# Autodesk Inventor assembly: Table
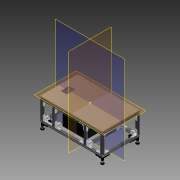
[picture p0: Inventor's stored thumbnail of the model, 180x180]
Saved by Autodesk Inventor 2015 (Build 190159000, 159)
## iProperties
Created: 2015-12-24
Part Number: Table
Document SubType Name: Assembly
Designer: Ryo
Author: Ryo
## Documents named in this file (10)
- D:\Users\Ryo\Documents\Inventor\motoman_cad\SIA5_TABLE\INVENTOR2015\Table_no_bis.iam
- D:\Users\Ryo\Documents\Inventor\motoman_table\EFS8-4040-580.ipt
- D:\Users\Ryo\Documents\Inventor\motoman_table\EFS8-4040-305.ipt
- D:\Users\Ryo\Documents\Inventor\motoman_cad\SIA5_TABLE\parts\EFS8-4040-1100.ipt
- D:\Users\Ryo\Documents\Inventor\motoman_cad\SIA5_TABLE\parts\SFK-N19T.ipt
- D:\Users\Ryo\Documents\Inventor\motoman_cad\SIA5_TABLE\INVENTOR2015\board.ipt
- D:\Users\Ryo\Documents\Inventor\motoman_cad\SIA5_TABLE\INVENTOR2015\controller_table.ipt
- D:\Users\Ryo\Documents\Inventor\motoman_cad\SIA5_TABLE\INVENTOR2015\controller.ipt
- D:\Users\Ryo\Documents\Inventor\Content Center Files\R2015\ja-JP\JIS B 1176\JIS B 1176 - M6 x 10.ipt
- D:\Users\Ryo\Documents\Inventor\motoman_cad\SIA5_TABLE\INVENTOR2015\foot_parts.iam
## Components (101 placed, 9 different names)
1. EFS8-4040-580:1 — フラッシュ:63, フラッシュ:64, メイト:70, フラッシュ:82, メイト:81, メイト:85, メイト:89, フラッシュ:86, メイト:91, フラッシュ:114
2. EFS8-4040-580:2 — フラッシュ:43, フラッシュ:44, メイト:44, フラッシュ:47, メイト:47, フラッシュ:49, メイト:51, フラッシュ:83, メイト:83, フラッシュ:89, メイト:95, フラッシュ:119, フラッシュ:122
3. EFS8-4040-580:4 — フラッシュ:16, メイト:26, フラッシュ:17, フラッシュ:18, フラッシュ:20, フラッシュ:54, メイト:62, フラッシュ:77, フラッシュ:78, フラッシュ:98, メイト:114, メイト:116, メイト:133
4. EFS8-4040-580:5 — フラッシュ:74, フラッシュ:75, メイト:73, フラッシュ:76, フラッシュ:95, メイト:108, フラッシュ:96, メイト:109, フラッシュ:101, メイト:119, フラッシュ:102, メイト:121
5. EFS8-4040-580:6 — フラッシュ:1, メイト:14, フラッシュ:2, フラッシュ:3, メイト:15, フラッシュ:4, フラッシュ:13, メイト:20, フラッシュ:15, メイト:24, フラッシュ:74, メイト:112, フラッシュ:100, メイト:117, フラッシュ:116, メイト:308, フラッシュ:118, メイト:309
6. EFS8-4040-580:7 — フラッシュ:68, メイト:72, フラッシュ:76, メイト:135, メイト:138, フラッシュ:111, メイト:140, フラッシュ:112, メイト:142
7. EFS8-4040-580:8 — フラッシュ:45, フラッシュ:46, メイト:45, フラッシュ:48, メイト:49, メイト:58, フラッシュ:52, メイト:74, フラッシュ:90, メイト:98, フラッシュ:91, メイト:100
8. EFS8-4040-305:1 — フラッシュ:18, フラッシュ:19, メイト:27, メイト:63, メイト:64, メイト:66, メイト:101, メイト:104
9. EFS8-4040-305:2 — フラッシュ:5, フラッシュ:6, メイト:16, メイト:18, フラッシュ:11, メイト:21, メイト:105, メイト:107
10. EFS8-4040-305:3 — フラッシュ:20, フラッシュ:21, メイト:28, メイト:34, メイト:36, フラッシュ:104, メイト:125, フラッシュ:105, メイト:128, メイト:134, フラッシュ:108
11. EFS8-4040-305:4 — フラッシュ:28, フラッシュ:29, メイト:32, メイト:42, メイト:46, フラッシュ:61, メイト:69, フラッシュ:62, メイト:90, メイト:94
12. EFS8-4040-305:5 — フラッシュ:7, フラッシュ:8, フラッシュ:9, メイト:17, メイト:22, メイト:25, メイト:120, フラッシュ:103, メイト:124
13. EFS8-4040-305:6 — フラッシュ:24, フラッシュ:25, メイト:30, フラッシュ:45, メイト:57, メイト:59, メイト:60, メイト:79, メイト:87
14. EFS8-4040-305:7 — フラッシュ:26, フラッシュ:27, メイト:31, メイト:50, メイト:52, メイト:54, フラッシュ:59, フラッシュ:60, メイト:68, メイト:78, メイト:82
15. EFS8-4040-305:8 — フラッシュ:22, フラッシュ:23, メイト:29, メイト:38, メイト:39, メイト:48, メイト:129, メイト:132
16. EFS8-4040-1100:1 — フラッシュ:3, メイト:15, フラッシュ:4, フラッシュ:7, フラッシュ:8, フラッシュ:9, メイト:17, フラッシュ:14, メイト:23, メイト:26, フラッシュ:17, フラッシュ:21, メイト:28, フラッシュ:22, フラッシュ:23, メイト:29, フラッシュ:28, フラッシュ:29, メイト:32, フラッシュ:30, メイト:33, メイト:35, フラッシュ:31, フラッシュ:32, メイト:37, フラッシュ:33, メイト:40, フラッシュ:42, メイト:43, フラッシュ:43, フラッシュ:44, フラッシュ:46, メイト:45, メイト:96, メイト:99, フラッシュ:99, メイト:115, メイト:118, フラッシュ:117, フラッシュ:120, メイト:310
17. EFS8-4040-1100:2 — フラッシュ:61, メイト:69, フラッシュ:62, フラッシュ:63, フラッシュ:68, メイト:72, フラッシュ:87, メイト:92, フラッシュ:88, メイト:93, メイト:122, メイト:123, メイト:126, メイト:127, フラッシュ:106, メイト:130, フラッシュ:107, メイト:131, メイト:139, メイト:141, メイト:307
18. EFS8-4040-1100:3 — フラッシュ:59, フラッシュ:60, メイト:68, フラッシュ:64, メイト:70, フラッシュ:75, メイト:73, フラッシュ:80, メイト:77, フラッシュ:81, メイト:80, フラッシュ:84, メイト:84, フラッシュ:85, メイト:88, フラッシュ:92, メイト:102, フラッシュ:93, メイト:103, フラッシュ:94, メイト:106, メイト:110, フラッシュ:109, メイト:136, フラッシュ:110, メイト:137, フラッシュ:113, メイト:313
19. EFS8-4040-1100:4 — フラッシュ:1, メイト:14, フラッシュ:2, フラッシュ:5, フラッシュ:6, メイト:16, フラッシュ:12, メイト:19, フラッシュ:16, フラッシュ:19, メイト:27, フラッシュ:24, フラッシュ:25, メイト:30, フラッシュ:26, フラッシュ:27, メイト:31, メイト:44, メイト:53, フラッシュ:51, メイト:56, フラッシュ:53, メイト:61, フラッシュ:55, メイト:65, フラッシュ:56, フラッシュ:57, メイト:67, フラッシュ:58, メイト:75, フラッシュ:79, メイト:86, メイト:97, フラッシュ:97, メイト:111, メイト:113, フラッシュ:115, フラッシュ:121, メイト:311
20. SFK-N19T:1 — フラッシュ:42, メイト:42, メイト:43
21. SFK-N19T:2 — フラッシュ:53, メイト:60, メイト:61
22. SFK-N19T:3 — フラッシュ:54, メイト:62, メイト:63
23. SFK-N19T:4 — フラッシュ:47, メイト:46, メイト:47
24. SFK-N19T:5 — フラッシュ:49, メイト:50, メイト:51, メイト:52
25. SFK-N19T:6 — メイト:58, フラッシュ:52, メイト:59
26. SFK-N19T:7 — フラッシュ:33, メイト:39, メイト:40
27. SFK-N19T:8 — メイト:35, フラッシュ:31, メイト:36
28. SFK-N19T:9 — フラッシュ:51, メイト:56, メイト:57
29. SFK-N19T:10 — フラッシュ:13, メイト:20, メイト:21
30. SFK-N19T:11 — メイト:53, メイト:54, フラッシュ:58
31. SFK-N19T:12 — フラッシュ:48, メイト:48, メイト:49
32. SFK-N19T:13 — フラッシュ:32, メイト:37, メイト:38
33. SFK-N19T:14 — フラッシュ:30, メイト:33, メイト:34
34. SFK-N19T:15 — メイト:18, フラッシュ:11, フラッシュ:12, メイト:19
35. SFK-N19T:16 — フラッシュ:15, メイト:24, メイト:25
36. SFK-N19T:17 — フラッシュ:55, メイト:64, メイト:65
37. SFK-N19T:18 — フラッシュ:14, メイト:22, メイト:23
38. SFK-N19T:19 — フラッシュ:56
39. SFK-N19T:20 — フラッシュ:57, メイト:66, メイト:67
40. board:1 — メイト:307, フラッシュ:113, フラッシュ:114, 挿入:125, 挿入:126, 挿入:127, 挿入:128, 挿入:129, 挿入:130, 挿入:131, 挿入:132, 挿入:133, 挿入:134, 挿入:135, 挿入:136, 挿入:137, 挿入:138, 挿入:139, 挿入:140, 挿入:141, 挿入:142, 挿入:143, 挿入:144, 挿入:145, 挿入:146, メイト:312, フラッシュ:123
41. controller_table:1 — メイト:74, メイト:75, フラッシュ:77, メイト:76
42. controller:1 — メイト:76, フラッシュ:78, フラッシュ:79
43. SFK-N19T:21 — フラッシュ:80, メイト:77, メイト:78
44. SFK-N19T:22 — フラッシュ:95, メイト:107, メイト:108
45. SFK-N19T:23 — フラッシュ:82, メイト:81, メイト:82
46. SFK-N19T:24 — フラッシュ:81, メイト:79, メイト:80
47. SFK-N19T:25 — フラッシュ:84, メイト:84, メイト:85
48. SFK-N19T:26 — フラッシュ:89, メイト:95, メイト:96
49. SFK-N19T:27 — フラッシュ:96, メイト:109, メイト:110
50. SFK-N19T:28 — フラッシュ:94, メイト:105, メイト:106
51. SFK-N19T:29 — フラッシュ:88, メイト:93, メイト:94
52. SFK-N19T:30 — メイト:89, フラッシュ:86, メイト:90
53. SFK-N19T:31 — フラッシュ:93, メイト:103, メイト:104
54. SFK-N19T:32 — フラッシュ:83, メイト:83, メイト:86
55. SFK-N19T:33 — フラッシュ:85, メイト:87, メイト:88
56. SFK-N19T:34 — フラッシュ:87, メイト:91, メイト:92
57. SFK-N19T:35 — フラッシュ:90, メイト:97, メイト:98
58. SFK-N19T:36 — フラッシュ:91, メイト:99, メイト:100
59. SFK-N19T:37 — フラッシュ:92, メイト:101, メイト:102
60. SFK-N19T:38 — フラッシュ:106, メイト:129, メイト:130
61. SFK-N19T:39 — フラッシュ:101, メイト:119, メイト:120
62. SFK-N19T:40 — フラッシュ:103, メイト:123, メイト:124
63. SFK-N19T:43 — メイト:139, フラッシュ:111, メイト:140
64. SFK-N19T:44 — フラッシュ:109, メイト:135, メイト:136
65. SFK-N19T:45 — フラッシュ:107, メイト:131, メイト:132
66. SFK-N19T:46 — フラッシュ:104, メイト:125, メイト:126
67. SFK-N19T:47 — フラッシュ:99, メイト:115, メイト:116
68. SFK-N19T:48 — フラッシュ:97, メイト:111, メイト:112
69. SFK-N19T:49 — フラッシュ:105, メイト:127, メイト:128
70. SFK-N19T:50 — フラッシュ:110, メイト:137, メイト:138
71. SFK-N19T:51 — メイト:133, メイト:134, フラッシュ:108
72. SFK-N19T:52 — フラッシュ:102, メイト:121, メイト:122
73. SFK-N19T:53 — フラッシュ:98, メイト:113, メイト:114
74. SFK-N19T:55 — フラッシュ:100, メイト:117, メイト:118
75. SFK-N19T:56 — フラッシュ:112, メイト:141, メイト:142
76. JIS B 1176 - メートル M6 x 10:1 — 挿入:125
77. JIS B 1176 - メートル M6 x 10:2 — 挿入:126
78. JIS B 1176 - メートル M6 x 10:3 — 挿入:127
79. JIS B 1176 - メートル M6 x 10:4 — 挿入:128
80. JIS B 1176 - メートル M6 x 10:5 — 挿入:129
81. JIS B 1176 - メートル M6 x 10:6 — 挿入:130
82. JIS B 1176 - メートル M6 x 10:7 — 挿入:131
83. JIS B 1176 - メートル M6 x 10:8 — 挿入:132
84. JIS B 1176 - メートル M6 x 10:9 — 挿入:133
85. JIS B 1176 - メートル M6 x 10:10 — 挿入:134
86. JIS B 1176 - メートル M6 x 10:11 — 挿入:135
87. JIS B 1176 - メートル M6 x 10:12 — 挿入:136
88. JIS B 1176 - メートル M6 x 10:13 — 挿入:137
89. JIS B 1176 - メートル M6 x 10:14 — 挿入:138
90. JIS B 1176 - メートル M6 x 10:15 — 挿入:139
91. JIS B 1176 - メートル M6 x 10:16 — 挿入:140
92. JIS B 1176 - メートル M6 x 10:17 — 挿入:141
93. JIS B 1176 - メートル M6 x 10:18 — 挿入:142
94. JIS B 1176 - メートル M6 x 10:19 — 挿入:143
95. JIS B 1176 - メートル M6 x 10:20 — 挿入:144
96. JIS B 1176 - メートル M6 x 10:21 — 挿入:145
97. JIS B 1176 - メートル M6 x 10:22 — 挿入:146
98. foot_parts:1 [sub-assembly] — フラッシュ:115, フラッシュ:116, メイト:308
99. foot_parts:2 [sub-assembly] — フラッシュ:117, フラッシュ:118, メイト:309
100. foot_parts:3 [sub-assembly] — フラッシュ:119, フラッシュ:120, メイト:310
101. foot_parts:4 [sub-assembly] — フラッシュ:121, フラッシュ:122, メイト:311
## Relationships (260: Mate 133, Flush 105, Insert 22)
- フラッシュ:1 [Flush]: EFS8-4040-580:6 ↔ EFS8-4040-1100:4
- メイト:14 [Mate]: EFS8-4040-580:6 ↔ EFS8-4040-1100:4
- フラッシュ:2 [Flush]: EFS8-4040-580:6 ↔ EFS8-4040-1100:4
- フラッシュ:3 [Flush]: EFS8-4040-580:6 ↔ EFS8-4040-1100:1
- メイト:15 [Mate]: EFS8-4040-580:6 ↔ EFS8-4040-1100:1
- フラッシュ:4 [Flush]: EFS8-4040-580:6 ↔ EFS8-4040-1100:1
- フラッシュ:5 [Flush]: EFS8-4040-305:2 ↔ EFS8-4040-1100:4
- フラッシュ:6 [Flush]: EFS8-4040-305:2 ↔ EFS8-4040-1100:4
- メイト:16 [Mate]: EFS8-4040-305:2 ↔ EFS8-4040-1100:4
- フラッシュ:7 [Flush]: EFS8-4040-305:5 ↔ EFS8-4040-1100:1
- フラッシュ:8 [Flush]: EFS8-4040-305:5 ↔ EFS8-4040-1100:1
- フラッシュ:9 [Flush]: EFS8-4040-305:5 ↔ EFS8-4040-1100:1
- メイト:17 [Mate]: EFS8-4040-305:5 ↔ EFS8-4040-1100:1
- メイト:18 [Mate]: EFS8-4040-305:2 ↔ SFK-N19T:15
- フラッシュ:11 [Flush] (5 mm): EFS8-4040-305:2 ↔ SFK-N19T:15
- フラッシュ:12 [Flush] (5 mm): EFS8-4040-1100:4 ↔ SFK-N19T:15
- メイト:19 [Mate]: EFS8-4040-1100:4 ↔ SFK-N19T:15
- フラッシュ:13 [Flush] (5 mm): EFS8-4040-580:6 ↔ SFK-N19T:10
- メイト:20 [Mate]: EFS8-4040-580:6 ↔ SFK-N19T:10
- メイト:21 [Mate]: EFS8-4040-305:2 ↔ SFK-N19T:10
- フラッシュ:14 [Flush] (5 mm): EFS8-4040-1100:1 ↔ SFK-N19T:18
- メイト:22 [Mate]: EFS8-4040-305:5 ↔ SFK-N19T:18
- メイト:23 [Mate]: EFS8-4040-1100:1 ↔ SFK-N19T:18
- フラッシュ:15 [Flush] (5 mm): EFS8-4040-580:6 ↔ SFK-N19T:16
- メイト:24 [Mate]: EFS8-4040-580:6 ↔ SFK-N19T:16
- メイト:25 [Mate]: EFS8-4040-305:5 ↔ SFK-N19T:16
- フラッシュ:16 [Flush] (295 mm): EFS8-4040-580:4 ↔ EFS8-4040-1100:4
- メイト:26 [Mate]: EFS8-4040-580:4 ↔ EFS8-4040-1100:1
- フラッシュ:17 [Flush]: EFS8-4040-580:4 ↔ EFS8-4040-1100:1
- フラッシュ:18 [Flush]: EFS8-4040-580:4 ↔ EFS8-4040-305:1
- フラッシュ:19 [Flush]: EFS8-4040-305:1 ↔ EFS8-4040-1100:4
- メイト:27 [Mate]: EFS8-4040-305:1 ↔ EFS8-4040-1100:4
- フラッシュ:20 [Flush]: EFS8-4040-580:4 ↔ EFS8-4040-305:3
- フラッシュ:21 [Flush]: EFS8-4040-305:3 ↔ EFS8-4040-1100:1
- メイト:28 [Mate]: EFS8-4040-305:3 ↔ EFS8-4040-1100:1
- フラッシュ:22 [Flush] (210 mm): EFS8-4040-305:8 ↔ EFS8-4040-1100:1
- フラッシュ:23 [Flush]: EFS8-4040-305:8 ↔ EFS8-4040-1100:1
- メイト:29 [Mate]: EFS8-4040-305:8 ↔ EFS8-4040-1100:1
- フラッシュ:24 [Flush] (210 mm): EFS8-4040-305:6 ↔ EFS8-4040-1100:4
- フラッシュ:25 [Flush]: EFS8-4040-305:6 ↔ EFS8-4040-1100:4
- メイト:30 [Mate]: EFS8-4040-305:6 ↔ EFS8-4040-1100:4
- フラッシュ:26 [Flush]: EFS8-4040-305:7 ↔ EFS8-4040-1100:4
- フラッシュ:27 [Flush]: EFS8-4040-305:7 ↔ EFS8-4040-1100:4
- メイト:31 [Mate]: EFS8-4040-305:7 ↔ EFS8-4040-1100:4
- フラッシュ:28 [Flush]: EFS8-4040-305:4 ↔ EFS8-4040-1100:1
- フラッシュ:29 [Flush]: EFS8-4040-305:4 ↔ EFS8-4040-1100:1
- メイト:32 [Mate]: EFS8-4040-305:4 ↔ EFS8-4040-1100:1
- フラッシュ:30 [Flush] (5 mm): EFS8-4040-1100:1 ↔ SFK-N19T:14
- メイト:33 [Mate]: EFS8-4040-1100:1 ↔ SFK-N19T:14
- メイト:34 [Mate]: EFS8-4040-305:3 ↔ SFK-N19T:14
- メイト:35 [Mate]: EFS8-4040-1100:1 ↔ SFK-N19T:8
- フラッシュ:31 [Flush] (5 mm): EFS8-4040-1100:1 ↔ SFK-N19T:8
- メイト:36 [Mate]: EFS8-4040-305:3 ↔ SFK-N19T:8
- フラッシュ:32 [Flush] (5 mm): EFS8-4040-1100:1 ↔ SFK-N19T:13
- メイト:37 [Mate]: EFS8-4040-1100:1 ↔ SFK-N19T:13
- メイト:38 [Mate]: EFS8-4040-305:8 ↔ SFK-N19T:13
- フラッシュ:33 [Flush] (5 mm): EFS8-4040-1100:1 ↔ SFK-N19T:7
- メイト:39 [Mate]: EFS8-4040-305:8 ↔ SFK-N19T:7
- メイト:40 [Mate]: EFS8-4040-1100:1 ↔ SFK-N19T:7
- フラッシュ:42 [Flush] (5 mm): EFS8-4040-1100:1 ↔ SFK-N19T:1
- メイト:42 [Mate]: EFS8-4040-305:4 ↔ SFK-N19T:1
- メイト:43 [Mate]: EFS8-4040-1100:1 ↔ SFK-N19T:1
- フラッシュ:43 [Flush]: EFS8-4040-580:2 ↔ EFS8-4040-1100:1
- フラッシュ:44 [Flush]: EFS8-4040-580:2 ↔ EFS8-4040-1100:1
- メイト:44 [Mate]: EFS8-4040-580:2 ↔ EFS8-4040-1100:4
- フラッシュ:45 [Flush]: EFS8-4040-580:8 ↔ EFS8-4040-305:6
- フラッシュ:46 [Flush]: EFS8-4040-580:8 ↔ EFS8-4040-1100:1
- メイト:45 [Mate]: EFS8-4040-580:8 ↔ EFS8-4040-1100:1
- フラッシュ:47 [Flush] (5 mm): EFS8-4040-580:2 ↔ SFK-N19T:4
- メイト:46 [Mate]: EFS8-4040-305:4 ↔ SFK-N19T:4
- メイト:47 [Mate]: EFS8-4040-580:2 ↔ SFK-N19T:4
- フラッシュ:48 [Flush] (5 mm): EFS8-4040-580:8 ↔ SFK-N19T:12
- メイト:48 [Mate]: EFS8-4040-305:8 ↔ SFK-N19T:12
- メイト:49 [Mate]: EFS8-4040-580:8 ↔ SFK-N19T:12
- フラッシュ:49 [Flush] (5 mm): EFS8-4040-580:2 ↔ SFK-N19T:5
- メイト:50 [Mate]: EFS8-4040-305:7 ↔ SFK-N19T:5
- メイト:51 [Mate]: EFS8-4040-580:2 ↔ SFK-N19T:5
- メイト:52 [Mate]: EFS8-4040-305:7 ↔ SFK-N19T:5
- メイト:53 [Mate]: EFS8-4040-1100:4 ↔ SFK-N19T:11
- メイト:54 [Mate]: EFS8-4040-305:7 ↔ SFK-N19T:11
- フラッシュ:51 [Flush] (5 mm): EFS8-4040-1100:4 ↔ SFK-N19T:9
- メイト:56 [Mate]: EFS8-4040-1100:4 ↔ SFK-N19T:9
- メイト:57 [Mate]: EFS8-4040-305:6 ↔ SFK-N19T:9
- メイト:58 [Mate]: EFS8-4040-580:8 ↔ SFK-N19T:6
- フラッシュ:52 [Flush] (5 mm): EFS8-4040-580:8 ↔ SFK-N19T:6
- メイト:59 [Mate]: EFS8-4040-305:6 ↔ SFK-N19T:6
- フラッシュ:53 [Flush] (5 mm): EFS8-4040-1100:4 ↔ SFK-N19T:2
- メイト:60 [Mate]: EFS8-4040-305:6 ↔ SFK-N19T:2
- メイト:61 [Mate]: EFS8-4040-1100:4 ↔ SFK-N19T:2
- フラッシュ:54 [Flush] (5 mm): EFS8-4040-580:4 ↔ SFK-N19T:3
- メイト:62 [Mate]: EFS8-4040-580:4 ↔ SFK-N19T:3
- メイト:63 [Mate]: EFS8-4040-305:1 ↔ SFK-N19T:3
- フラッシュ:55 [Flush] (5 mm): EFS8-4040-1100:4 ↔ SFK-N19T:17
- メイト:64 [Mate]: EFS8-4040-305:1 ↔ SFK-N19T:17
- メイト:65 [Mate]: EFS8-4040-1100:4 ↔ SFK-N19T:17
- フラッシュ:56 [Flush] (5 mm): EFS8-4040-1100:4 ↔ SFK-N19T:19
- フラッシュ:57 [Flush] (5 mm): EFS8-4040-1100:4 ↔ SFK-N19T:20
- メイト:66 [Mate]: EFS8-4040-305:1 ↔ SFK-N19T:20
- メイト:67 [Mate]: EFS8-4040-1100:4 ↔ SFK-N19T:20
- フラッシュ:58 [Flush] (5 mm): EFS8-4040-1100:4 ↔ SFK-N19T:11
- フラッシュ:59 [Flush]: EFS8-4040-305:7 ↔ EFS8-4040-1100:3
- フラッシュ:60 [Flush]: EFS8-4040-305:7 ↔ EFS8-4040-1100:3
- メイト:68 [Mate]: EFS8-4040-305:7 ↔ EFS8-4040-1100:3
- フラッシュ:61 [Flush]: EFS8-4040-305:4 ↔ EFS8-4040-1100:2
- メイト:69 [Mate]: EFS8-4040-305:4 ↔ EFS8-4040-1100:2
- フラッシュ:62 [Flush]: EFS8-4040-305:4 ↔ EFS8-4040-1100:2
- フラッシュ:63 [Flush]: EFS8-4040-580:1 ↔ EFS8-4040-1100:2
- フラッシュ:64 [Flush]: EFS8-4040-580:1 ↔ EFS8-4040-1100:3
- メイト:70 [Mate]: EFS8-4040-580:1 ↔ EFS8-4040-1100:3
- フラッシュ:68 [Flush]: EFS8-4040-580:7 ↔ EFS8-4040-1100:2
- メイト:72 [Mate]: EFS8-4040-580:7 ↔ EFS8-4040-1100:2
- フラッシュ:74 [Flush]: EFS8-4040-580:5 ↔ EFS8-4040-580:6
- フラッシュ:75 [Flush]: EFS8-4040-580:5 ↔ EFS8-4040-1100:3
- メイト:73 [Mate]: EFS8-4040-580:5 ↔ EFS8-4040-1100:3
- フラッシュ:76 [Flush] (530 mm): EFS8-4040-580:5 ↔ EFS8-4040-580:7
- メイト:74 [Mate]: EFS8-4040-580:8 ↔ controller_table:1
- メイト:75 [Mate]: EFS8-4040-1100:4 ↔ controller_table:1
- フラッシュ:77 [Flush]: EFS8-4040-580:4 ↔ controller_table:1
- メイト:76 [Mate]: controller_table:1 ↔ controller:1
- フラッシュ:78 [Flush] (-87.5 mm): EFS8-4040-580:4 ↔ controller:1
- フラッシュ:79 [Flush] (95 mm): EFS8-4040-1100:4 ↔ controller:1
- フラッシュ:80 [Flush] (5 mm): EFS8-4040-1100:3 ↔ SFK-N19T:21
- メイト:77 [Mate]: EFS8-4040-1100:3 ↔ SFK-N19T:21
- メイト:78 [Mate]: EFS8-4040-305:7 ↔ SFK-N19T:21
- フラッシュ:81 [Flush] (5 mm): EFS8-4040-1100:3 ↔ SFK-N19T:24
- メイト:79 [Mate]: EFS8-4040-305:6 ↔ SFK-N19T:24
- メイト:80 [Mate]: EFS8-4040-1100:3 ↔ SFK-N19T:24
- フラッシュ:82 [Flush] (5 mm): EFS8-4040-580:1 ↔ SFK-N19T:23
- メイト:81 [Mate]: EFS8-4040-580:1 ↔ SFK-N19T:23
- メイト:82 [Mate]: EFS8-4040-305:7 ↔ SFK-N19T:23
- フラッシュ:83 [Flush] (5 mm): EFS8-4040-580:2 ↔ SFK-N19T:32
- メイト:83 [Mate]: EFS8-4040-580:2 ↔ SFK-N19T:32
- フラッシュ:84 [Flush] (5 mm): EFS8-4040-1100:3 ↔ SFK-N19T:25
- メイト:84 [Mate]: EFS8-4040-1100:3 ↔ SFK-N19T:25
- メイト:85 [Mate]: EFS8-4040-580:1 ↔ SFK-N19T:25
- メイト:86 [Mate]: EFS8-4040-1100:4 ↔ SFK-N19T:32
- フラッシュ:85 [Flush] (5 mm): EFS8-4040-1100:3 ↔ SFK-N19T:33
- メイト:87 [Mate]: EFS8-4040-305:6 ↔ SFK-N19T:33
- メイト:88 [Mate]: EFS8-4040-1100:3 ↔ SFK-N19T:33
- メイト:89 [Mate]: EFS8-4040-580:1 ↔ SFK-N19T:30
- フラッシュ:86 [Flush] (5 mm): EFS8-4040-580:1 ↔ SFK-N19T:30
- メイト:90 [Mate]: EFS8-4040-305:4 ↔ SFK-N19T:30
- フラッシュ:87 [Flush] (5 mm): EFS8-4040-1100:2 ↔ SFK-N19T:34
- メイト:91 [Mate]: EFS8-4040-580:1 ↔ SFK-N19T:34
- メイト:92 [Mate]: EFS8-4040-1100:2 ↔ SFK-N19T:34
- フラッシュ:88 [Flush] (5 mm): EFS8-4040-1100:2 ↔ SFK-N19T:29
- メイト:93 [Mate]: EFS8-4040-1100:2 ↔ SFK-N19T:29
- メイト:94 [Mate]: EFS8-4040-305:4 ↔ SFK-N19T:29
- フラッシュ:89 [Flush] (5 mm): EFS8-4040-580:2 ↔ SFK-N19T:26
- メイト:95 [Mate]: EFS8-4040-580:2 ↔ SFK-N19T:26
- メイト:96 [Mate]: EFS8-4040-1100:1 ↔ SFK-N19T:26
- フラッシュ:90 [Flush] (5 mm): EFS8-4040-580:8 ↔ SFK-N19T:35
- メイト:97 [Mate]: EFS8-4040-1100:4 ↔ SFK-N19T:35
- メイト:98 [Mate]: EFS8-4040-580:8 ↔ SFK-N19T:35
- フラッシュ:91 [Flush] (5 mm): EFS8-4040-580:8 ↔ SFK-N19T:36
- メイト:99 [Mate]: EFS8-4040-1100:1 ↔ SFK-N19T:36
- メイト:100 [Mate]: EFS8-4040-580:8 ↔ SFK-N19T:36
- フラッシュ:92 [Flush] (5 mm): EFS8-4040-1100:3 ↔ SFK-N19T:37
- メイト:101 [Mate]: EFS8-4040-305:1 ↔ SFK-N19T:37
- メイト:102 [Mate]: EFS8-4040-1100:3 ↔ SFK-N19T:37
- フラッシュ:93 [Flush]: EFS8-4040-1100:3 ↔ SFK-N19T:31
- メイト:103 [Mate]: EFS8-4040-1100:3 ↔ SFK-N19T:31
- メイト:104 [Mate]: EFS8-4040-305:1 ↔ SFK-N19T:31
- フラッシュ:94 [Flush] (5 mm): EFS8-4040-1100:3 ↔ SFK-N19T:28
- メイト:105 [Mate]: EFS8-4040-305:2 ↔ SFK-N19T:28
- メイト:106 [Mate]: EFS8-4040-1100:3 ↔ SFK-N19T:28
- フラッシュ:95 [Flush] (5 mm): EFS8-4040-580:5 ↔ SFK-N19T:22
- メイト:107 [Mate]: EFS8-4040-305:2 ↔ SFK-N19T:22
- メイト:108 [Mate]: EFS8-4040-580:5 ↔ SFK-N19T:22
- フラッシュ:96 [Flush]: EFS8-4040-580:5 ↔ SFK-N19T:27
- メイト:109 [Mate]: EFS8-4040-580:5 ↔ SFK-N19T:27
- メイト:110 [Mate]: EFS8-4040-1100:3 ↔ SFK-N19T:27
- フラッシュ:97 [Flush] (5 mm): EFS8-4040-1100:4 ↔ SFK-N19T:48
- メイト:111 [Mate]: EFS8-4040-1100:4 ↔ SFK-N19T:48
- メイト:112 [Mate]: EFS8-4040-580:6 ↔ SFK-N19T:48
- フラッシュ:98 [Flush] (5 mm): EFS8-4040-580:4 ↔ SFK-N19T:53
- メイト:113 [Mate]: EFS8-4040-1100:4 ↔ SFK-N19T:53
- メイト:114 [Mate]: EFS8-4040-580:4 ↔ SFK-N19T:53
- フラッシュ:99 [Flush] (5 mm): EFS8-4040-1100:1 ↔ SFK-N19T:47
- メイト:115 [Mate]: EFS8-4040-1100:1 ↔ SFK-N19T:47
- メイト:116 [Mate]: EFS8-4040-580:4 ↔ SFK-N19T:47
- フラッシュ:100 [Flush] (5 mm): EFS8-4040-580:6 ↔ SFK-N19T:55
- メイト:117 [Mate]: EFS8-4040-580:6 ↔ SFK-N19T:55
- メイト:118 [Mate]: EFS8-4040-1100:1 ↔ SFK-N19T:55
- フラッシュ:101 [Flush] (5 mm): EFS8-4040-580:5 ↔ SFK-N19T:39
- メイト:119 [Mate]: EFS8-4040-580:5 ↔ SFK-N19T:39
- メイト:120 [Mate]: EFS8-4040-305:5 ↔ SFK-N19T:39
- フラッシュ:102 [Flush] (5 mm): EFS8-4040-580:5 ↔ SFK-N19T:52
- メイト:121 [Mate]: EFS8-4040-580:5 ↔ SFK-N19T:52
- メイト:122 [Mate]: EFS8-4040-1100:2 ↔ SFK-N19T:52
- フラッシュ:103 [Flush]: EFS8-4040-305:5 ↔ SFK-N19T:40
- メイト:123 [Mate]: EFS8-4040-1100:2 ↔ SFK-N19T:40
- メイト:124 [Mate]: EFS8-4040-305:5 ↔ SFK-N19T:40
- フラッシュ:104 [Flush]: EFS8-4040-305:3 ↔ SFK-N19T:46
- メイト:125 [Mate]: EFS8-4040-305:3 ↔ SFK-N19T:46
- メイト:126 [Mate]: EFS8-4040-1100:2 ↔ SFK-N19T:46
- フラッシュ:105 [Flush] (5 mm): EFS8-4040-305:3 ↔ SFK-N19T:49
- メイト:127 [Mate]: EFS8-4040-1100:2 ↔ SFK-N19T:49
- メイト:128 [Mate]: EFS8-4040-305:3 ↔ SFK-N19T:49
- フラッシュ:106 [Flush] (5 mm): EFS8-4040-1100:2 ↔ SFK-N19T:38
- メイト:129 [Mate]: EFS8-4040-305:8 ↔ SFK-N19T:38
- メイト:130 [Mate]: EFS8-4040-1100:2 ↔ SFK-N19T:38
- フラッシュ:107 [Flush] (5 mm): EFS8-4040-1100:2 ↔ SFK-N19T:45
- メイト:131 [Mate]: EFS8-4040-1100:2 ↔ SFK-N19T:45
- メイト:132 [Mate]: EFS8-4040-305:8 ↔ SFK-N19T:45
- メイト:133 [Mate]: EFS8-4040-580:4 ↔ SFK-N19T:51
- メイト:134 [Mate]: EFS8-4040-305:3 ↔ SFK-N19T:51
- フラッシュ:108 [Flush] (5 mm): EFS8-4040-305:3 ↔ SFK-N19T:51
- フラッシュ:109 [Flush] (5 mm): EFS8-4040-1100:3 ↔ SFK-N19T:44
- メイト:135 [Mate]: EFS8-4040-580:7 ↔ SFK-N19T:44
- メイト:136 [Mate]: EFS8-4040-1100:3 ↔ SFK-N19T:44
- フラッシュ:110 [Flush] (5 mm): EFS8-4040-1100:3 ↔ SFK-N19T:50
- メイト:137 [Mate]: EFS8-4040-1100:3 ↔ SFK-N19T:50
- メイト:138 [Mate]: EFS8-4040-580:7 ↔ SFK-N19T:50
- メイト:139 [Mate]: EFS8-4040-1100:2 ↔ SFK-N19T:43
- フラッシュ:111 [Flush] (5 mm): EFS8-4040-580:7 ↔ SFK-N19T:43
- メイト:140 [Mate]: EFS8-4040-580:7 ↔ SFK-N19T:43
- フラッシュ:112 [Flush] (5 mm): EFS8-4040-580:7 ↔ SFK-N19T:56
- メイト:141 [Mate]: EFS8-4040-1100:2 ↔ SFK-N19T:56
- メイト:142 [Mate]: EFS8-4040-580:7 ↔ SFK-N19T:56
- メイト:307 [Mate]: EFS8-4040-1100:2 ↔ board:1
- フラッシュ:113 [Flush]: EFS8-4040-1100:3 ↔ board:1
- フラッシュ:114 [Flush]: EFS8-4040-580:1 ↔ board:1
- 挿入:125 [Insert]: board:1 ↔ JIS B 1176 - メートル M6 x 10:1
- 挿入:126 [Insert]: board:1 ↔ JIS B 1176 - メートル M6 x 10:2
- 挿入:127 [Insert]: board:1 ↔ JIS B 1176 - メートル M6 x 10:3
- 挿入:128 [Insert]: board:1 ↔ JIS B 1176 - メートル M6 x 10:4
- 挿入:129 [Insert]: board:1 ↔ JIS B 1176 - メートル M6 x 10:5
- 挿入:130 [Insert]: board:1 ↔ JIS B 1176 - メートル M6 x 10:6
- 挿入:131 [Insert]: board:1 ↔ JIS B 1176 - メートル M6 x 10:7
- 挿入:132 [Insert]: board:1 ↔ JIS B 1176 - メートル M6 x 10:8
- 挿入:133 [Insert]: board:1 ↔ JIS B 1176 - メートル M6 x 10:9
- 挿入:134 [Insert]: board:1 ↔ JIS B 1176 - メートル M6 x 10:10
- 挿入:135 [Insert]: board:1 ↔ JIS B 1176 - メートル M6 x 10:11
- 挿入:136 [Insert]: board:1 ↔ JIS B 1176 - メートル M6 x 10:12
- 挿入:137 [Insert]: board:1 ↔ JIS B 1176 - メートル M6 x 10:13
- 挿入:138 [Insert]: board:1 ↔ JIS B 1176 - メートル M6 x 10:14
- 挿入:139 [Insert]: board:1 ↔ JIS B 1176 - メートル M6 x 10:15
- 挿入:140 [Insert]: board:1 ↔ JIS B 1176 - メートル M6 x 10:16
- 挿入:141 [Insert]: board:1 ↔ JIS B 1176 - メートル M6 x 10:17
- 挿入:142 [Insert]: board:1 ↔ JIS B 1176 - メートル M6 x 10:18
- 挿入:143 [Insert]: board:1 ↔ JIS B 1176 - メートル M6 x 10:19
- 挿入:144 [Insert]: board:1 ↔ JIS B 1176 - メートル M6 x 10:20
- 挿入:145 [Insert]: board:1 ↔ JIS B 1176 - メートル M6 x 10:21
- 挿入:146 [Insert]: board:1 ↔ JIS B 1176 - メートル M6 x 10:22
- フラッシュ:115 [Flush]: EFS8-4040-1100:4 ↔ foot_parts:1
- フラッシュ:116 [Flush]: EFS8-4040-580:6 ↔ foot_parts:1
- メイト:308 [Mate]: EFS8-4040-580:6 ↔ foot_parts:1
- フラッシュ:117 [Flush]: EFS8-4040-1100:1 ↔ foot_parts:2
- フラッシュ:118 [Flush]: EFS8-4040-580:6 ↔ foot_parts:2
- メイト:309 [Mate]: EFS8-4040-580:6 ↔ foot_parts:2
- フラッシュ:119 [Flush]: EFS8-4040-580:2 ↔ foot_parts:3
- フラッシュ:120 [Flush]: EFS8-4040-1100:1 ↔ foot_parts:3
- メイト:310 [Mate]: EFS8-4040-1100:1 ↔ foot_parts:3
- フラッシュ:121 [Flush]: EFS8-4040-1100:4 ↔ foot_parts:4
- フラッシュ:122 [Flush]: EFS8-4040-580:2 ↔ foot_parts:4
- メイト:311 [Mate]: EFS8-4040-1100:4 ↔ foot_parts:4
- メイト:312 [Mate] (-550 mm): board:1
- フラッシュ:123 [Flush]: board:1
- メイト:313 [Mate] (-330 mm): EFS8-4040-1100:3
